# Autodesk Inventor assembly: protoswitchboard
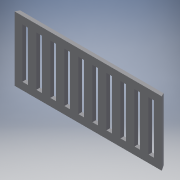
[picture p0: Inventor's stored thumbnail of the model, 180x180]
Saved by Autodesk Inventor 2017 (Build 210142000, 142)
## iProperties
Created: 2017-08-24
Part Number: protoswitchboard
Document SubType Name: Assembly
Designer: erwin
Author: erwin
## Documents named in this file (3)
- D:\GitHub\ProtoSwitchBoard\2\protoswitchboard.iam
- D:\GitHub\ProtoSwitchBoard\2\pcbcover.ipt
- D:\GitHub\ProtoSwitchBoard\2\base.ipt
## Components (2 placed, 2 different names)
1. pcbcover:1 — Flush:1
2. base:1 — Flush:1
## Relationships (1: Flush 1)
- Flush:1: pcbcover:1 ↔ base:1
